# Autodesk Inventor assembly: ASY Beshkino_bio_tank
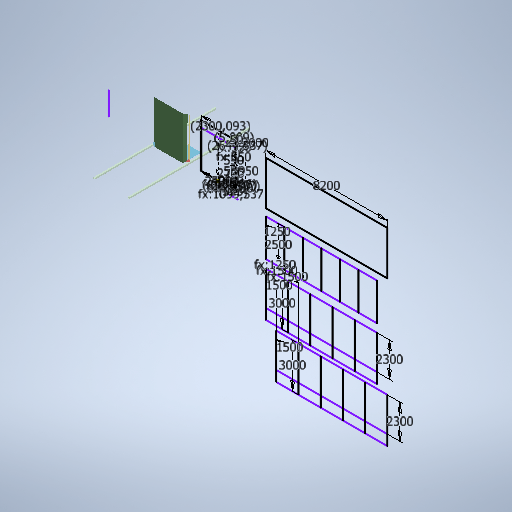
[picture p0: Inventor's stored thumbnail of the model, 512x512]
Saved by Autodesk Inventor 2025 (Build 290162010, 162A)
## iProperties
Created: 2024-07-21
Part Number: ASY Beshkino_bio_tank
Document SubType Name: Assembly
Designer: admin
Author: admin
## Documents named in this file (7)
- C:\Users\user\YandexDisk\домашниий пк\Inventor\BSH_Beshkino_bio_tank\ASY Beshkino_bio_tank.iam
- C:\Users\user\YandexDisk\домашниий пк\Inventor\BSH_Beshkino_bio_tank\BSH 000 dim Beshkino_bio_tank.ipt
- C:\Users\user\YandexDisk\домашниий пк\Inventor\BSH_Beshkino_bio_tank\BSH 010 floor 1.ipt
- C:\Users\user\YandexDisk\домашниий пк\Inventor\BSH_Beshkino_bio_tank\BSH 021 rib 1.ipt
- C:\Users\user\YandexDisk\домашниий пк\Inventor\BSH_Beshkino_bio_tank\BSH 022 rib 2.ipt
- C:\Users\user\YandexDisk\домашниий пк\Inventor\BSH_Beshkino_bio_tank\BSH 061 tube 1.ipt
- C:\Users\user\YandexDisk\домашниий пк\Inventor\BSH_Beshkino_bio_tank\BSH 031 nose 1.ipt
## Components (8 placed, 6 different names)
1. BSH 000 dim Beshkino_bio_tank:1
2. BSH 010 floor 1:1 — Mate:5, Mate:6, Mate:7
3. BSH 020 rib 1:1 — Flush:2, Mate:4, Flush:3, Mate:5, Mate:6, Rigid:2, Rigid:3
4. BSH 022 rib 2:1 — Rigid:3
5. BSH 061 tube 1:1 — Mate:1, Rigid:1, Mate:3
6. BSH 061 tube 1:2 — Mate:2, Rigid:1, Mate:4, Flush:3
7. BSH 020 rib 1:2 — Rigid:2
8. BSH 031 nose 1:1 — Mate:7
## Relationships (12: Mate 7, WeldJoint 3, Flush 2)
- Flush:2: BSH 020 rib 1:1
- Mate:1: BSH 061 tube 1:1
- Mate:2: BSH 061 tube 1:2
- Rigid:1 [WeldJoint] (-2400 mm): BSH 061 tube 1:1 ↔ BSH 061 tube 1:2
- Mate:3: BSH 061 tube 1:1
- Mate:4: BSH 020 rib 1:1 ↔ BSH 061 tube 1:2
- Flush:3: BSH 020 rib 1:1 ↔ BSH 061 tube 1:2
- Mate:5: BSH 010 floor 1:1 ↔ BSH 020 rib 1:1
- Mate:6: BSH 010 floor 1:1 ↔ BSH 020 rib 1:1
- Rigid:2 [WeldJoint]: BSH 020 rib 1:1 ↔ BSH 020 rib 1:2
- Rigid:3 [WeldJoint]: BSH 020 rib 1:1 ↔ BSH 022 rib 2:1
- Mate:7: BSH 010 floor 1:1 ↔ BSH 031 nose 1:1
